# Autodesk Inventor assembly: Jar Jar
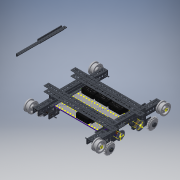
[picture p0: Inventor's stored thumbnail of the model, 180x180]
Saved by Autodesk Inventor 2016 (Build 200138000, 138)
## iProperties
Created: 2015-12-13
Part Number: Jar Jar
Document SubType Name: Assembly
Designer: tbloo
Author: tbloo
## Documents named in this file (19)
- C:\Users\TimB\Documents\GitHub\phi_robotics\3d-models\FTC_Tetrix_KOP_Block_Party\Tim Bloot Designs\JAr JaR Bot\Jar Jar.iam
- C:\Users\TimB\Documents\GitHub\phi_robotics\3d-models\FTC_Tetrix_KOP_Block_Party\Tim Bloot Designs\Base Plate.ipt
- C:\Users\TimB\Documents\GitHub\phi_robotics\3d-models\FTC_Tetrix_KOP_Block_Party\Tetrix_Kit_FTC\Autodesk Inventor Files\tetrix_c_channel-3.ipt
- C:\Users\TimB\Documents\GitHub\phi_robotics\3d-models\FTC_Tetrix_KOP_Block_Party\Tetrix_Kit_FTC\Autodesk Inventor Files\tetrix_c_channel-2.ipt
- C:\Users\TimB\Documents\GitHub\phi_robotics\3d-models\FTC_Tetrix_KOP_Block_Party\Tetrix_Kit_FTC\Autodesk Inventor Files\tetrix_motor_mount-old.ipt
- C:\Users\TimB\Documents\GitHub\phi_robotics\3d-models\FTC_Tetrix_KOP_Block_Party\Tetrix_Kit_FTC\Autodesk Inventor Files\tetrix_motor.iam
- C:\Users\TimB\Documents\GitHub\phi_robotics\3d-models\FTC_Tetrix_KOP_Block_Party\Tetrix_Kit_FTC\Autodesk Inventor Files\tetrix_bushing.ipt
- C:\Users\TimB\Documents\GitHub\phi_robotics\3d-models\FTC_Tetrix_KOP_Block_Party\Tim Bloot Designs\JAr JaR Bot\Tread Wheel Assembly.iam
- C:\Users\TimB\Documents\GitHub\phi_robotics\3d-models\FTC_Tetrix_KOP_Block_Party\Tetrix_Kit_FTC\Autodesk Inventor Files\tetrix_c_channel-5.ipt
- C:\Users\TimB\Documents\GitHub\phi_robotics\3d-models\FTC_Tetrix_KOP_Block_Party\Tetrix_Kit_FTC\Autodesk Inventor Files\tetrix_inside_corner_bracket.ipt
- C:\Users\TimB\Documents\GitHub\phi_robotics\3d-models\FTC_Tetrix_KOP_Block_Party\Tetrix_Kit_FTC\Autodesk Inventor Files\tetrix_motor_controller.ipt
- C:\Users\TimB\Documents\GitHub\phi_robotics\3d-models\FTC_Tetrix_KOP_Block_Party\Tetrix_Kit_FTC\Autodesk Inventor Files\tetrix_servo_controller.ipt
- C:\Users\TimB\Documents\GitHub\phi_robotics\3d-models\FTC_Tetrix_KOP_Block_Party\Tetrix_Kit_FTC\Autodesk Inventor Files\tetrix_c_channel-round.ipt
- C:\Users\TimB\Documents\GitHub\phi_robotics\3d-models\FTC_Tetrix_KOP_Block_Party\Tetrix_Kit_FTC\Autodesk Inventor Files\tetrix_c_channel-1.ipt
- C:\Users\TimB\Documents\GitHub\phi_robotics\3d-models\FTC_Tetrix_KOP_Block_Party\Tetrix_Kit_FTC\Autodesk Inventor Files\tetrix_angle-288 MM.ipt
- C:\Users\TimB\Documents\GitHub\phi_robotics\3d-models\FTC_Tetrix_KOP_Block_Party\Tim Bloot Designs\JAr JaR Bot\Tread Sproket Gear Assembly 2.iam
- C:\Users\TimB\Documents\GitHub\phi_robotics\3d-models\FTC_Tetrix_KOP_Block_Party\Tetrix_Kit_FTC\Autodesk Inventor Files\tetrix_739274_2013.ipt
- C:\Users\TimB\Documents\GitHub\phi_robotics\3d-models\FTC_Tetrix_KOP_Block_Party\Tim Bloot Designs\JAr JaR Bot\Motor Med Chain gear.iam
- C:\Users\TimB\Documents\GitHub\phi_robotics\3d-models\FTC_Tetrix_KOP_Block_Party\Tetrix_Kit_FTC\Autodesk Inventor Files\tetrix_angle-144 MM.ipt
## Components (61 placed, 18 different names)
1. Base Plate:1 — Rigid:60, Rigid:61, Rigid:63, Rigid:85, Rigid:108
2. tetrix_c_channel-3:4 — Rigid:55, Rigid:56, Rigid:76, Rigid:110
3. tetrix_c_channel-2:13 — Rigid:64, Rigid:86, Rigid:111
4. tetrix_c_channel-2:15 — Rigid:109
5. tetrix_c_channel-2:16
6. tetrix_motor_mount-old:6
7. tetrix_motor:5 [sub-assembly] — Rigid:91
8. Tread Wheel Assembly:5 [sub-assembly]
9. Tread Wheel Assembly:6 [sub-assembly]
10. tetrix_c_channel-5:1 — Rigid:55
11. tetrix_c_channel-5:2 — Rigid:59
12. tetrix_inside_corner_bracket:2 — Rigid:56, Rigid:59
13. tetrix_motor_controller:1 — Rigid:61, Rigid:62
14. tetrix_motor_controller:2 — Rigid:60
15. tetrix_motor_controller:3 — Rigid:62
16. tetrix_servo_controller:1 — Rigid:63
17. tetrix_c_channel-round:1 — Rigid:64, Rigid:65
18. tetrix_c_channel-1:1 — Rigid:65, Rotational:33, Rotational:34
19. tetrix_bushing:13 — Rotational:33, Rotational:42
20. tetrix_bushing:14 — Rotational:34
21. tetrix_c_channel-2:18 — Rigid:75
22. tetrix_motor_mount-old:8 — Rotational:41
23. tetrix_c_channel-round:3
24. tetrix_c_channel-1:3
25. tetrix_bushing:17
26. tetrix_bushing:18 — Rotational:43
27. tetrix_angle-288 MM:2 — Rigid:75, Rigid:76, Rigid:85, Rigid:86
28. tetrix_motor:6 [sub-assembly] — Rotational:41, Rigid:92
29. Tread Sproket Gear Assembly 2:1 [sub-assembly] — Rotational:42
30. Tread Sproket Gear Assembly 2:2 [sub-assembly] — Rotational:43
31. Motor Med Chain gear:1 [sub-assembly] — Rigid:92
32. Motor Med Chain gear:2 [sub-assembly] — Rigid:91
33. tetrix_c_channel-3:5
34. tetrix_c_channel-2:19
35. tetrix_c_channel-2:20
36. tetrix_c_channel-2:21
37. tetrix_motor_mount-old:9
38. tetrix_motor:7 [sub-assembly]
39. Tread Wheel Assembly:7 [sub-assembly]
40. Tread Wheel Assembly:8 [sub-assembly]
41. tetrix_c_channel-round:4
42. tetrix_c_channel-1:4
43. tetrix_bushing:19
44. tetrix_bushing:20
45. tetrix_c_channel-2:22
46. tetrix_motor_mount-old:10
47. tetrix_c_channel-round:5
48. tetrix_c_channel-1:5
49. tetrix_bushing:21
50. tetrix_bushing:22
51. tetrix_angle-288 MM:3 — Rigid:108
52. tetrix_motor:8 [sub-assembly]
53. Tread Sproket Gear Assembly 2:3 [sub-assembly]
54. Tread Sproket Gear Assembly 2:4 [sub-assembly]
55. tetrix_739274_2013:3
56. tetrix_739274_2013:4
57. Motor Med Chain gear:3 [sub-assembly]
58. Motor Med Chain gear:4 [sub-assembly]
59. tetrix_angle-288 MM:4
60. tetrix_angle-144 MM:1 — Rigid:109, Rigid:110, Rigid:111
61. tetrix_angle-144 MM:2
## Relationships (58: WeldJoint 38, RevoluteJoint 20)
- [WeldJoint]: tetrix_c_channel-2:13 ↔ tetrix_motor_mount-old:6
- [RevoluteJoint]: tetrix_motor_mount-old:6 ↔ tetrix_motor:5
- [RevoluteJoint]: tetrix_c_channel-2:15 ↔ Tread Wheel Assembly:5
- [RevoluteJoint]: tetrix_c_channel-2:16 ↔ Tread Wheel Assembly:6
- Rigid:55 [WeldJoint]: tetrix_c_channel-3:4 ↔ tetrix_c_channel-5:1
- Rigid:56 [WeldJoint]: tetrix_c_channel-3:4 ↔ tetrix_inside_corner_bracket:2
- Rigid:59 [WeldJoint]: tetrix_c_channel-5:2 ↔ tetrix_inside_corner_bracket:2
- Rigid:60 [WeldJoint]: Base Plate:1 ↔ tetrix_motor_controller:2
- Rigid:61 [WeldJoint]: Base Plate:1 ↔ tetrix_motor_controller:1
- Rigid:62 [WeldJoint]: tetrix_motor_controller:1 ↔ tetrix_motor_controller:3
- Rigid:63 [WeldJoint]: Base Plate:1 ↔ tetrix_servo_controller:1
- Rigid:64 [WeldJoint]: tetrix_c_channel-2:13 ↔ tetrix_c_channel-round:1
- Rigid:65 [WeldJoint]: tetrix_c_channel-round:1 ↔ tetrix_c_channel-1:1
- Rotational:33 [RevoluteJoint]: tetrix_c_channel-1:1 ↔ tetrix_bushing:13
- Rotational:34 [RevoluteJoint]: tetrix_c_channel-1:1 ↔ tetrix_bushing:14
- [WeldJoint]: tetrix_c_channel-2:18 ↔ tetrix_motor_mount-old:8
- [WeldJoint]: tetrix_c_channel-2:18 ↔ tetrix_c_channel-round:3
- [WeldJoint]: tetrix_c_channel-round:3 ↔ tetrix_c_channel-1:3
- [RevoluteJoint]: tetrix_c_channel-1:3 ↔ tetrix_bushing:17
- [RevoluteJoint]: tetrix_c_channel-1:3 ↔ tetrix_bushing:18
- Rigid:75 [WeldJoint]: tetrix_c_channel-2:18 ↔ tetrix_angle-288 MM:2
- Rigid:76 [WeldJoint]: tetrix_c_channel-3:4 ↔ tetrix_angle-288 MM:2
- Rotational:41 [RevoluteJoint]: tetrix_motor_mount-old:8 ↔ tetrix_motor:6
- Rotational:42 [RevoluteJoint]: tetrix_bushing:13 ↔ Tread Sproket Gear Assembly 2:1
- Rotational:43 [RevoluteJoint]: tetrix_bushing:18 ↔ Tread Sproket Gear Assembly 2:2
- Rigid:85 [WeldJoint]: Base Plate:1 ↔ tetrix_angle-288 MM:2
- Rigid:86 [WeldJoint]: tetrix_c_channel-2:13 ↔ tetrix_angle-288 MM:2
- Rigid:91 [WeldJoint]: tetrix_motor:5 ↔ Motor Med Chain gear:2
- Rigid:92 [WeldJoint]: tetrix_motor:6 ↔ Motor Med Chain gear:1
- [WeldJoint]: tetrix_c_channel-2:19 ↔ tetrix_motor_mount-old:9
- [RevoluteJoint]: tetrix_motor_mount-old:9 ↔ tetrix_motor:7
- [RevoluteJoint]: tetrix_c_channel-2:20 ↔ Tread Wheel Assembly:7
- [RevoluteJoint]: tetrix_c_channel-2:21 ↔ Tread Wheel Assembly:8
- [WeldJoint]: tetrix_c_channel-2:19 ↔ tetrix_c_channel-round:4
- [WeldJoint]: tetrix_c_channel-round:4 ↔ tetrix_c_channel-1:4
- [RevoluteJoint]: tetrix_c_channel-1:4 ↔ tetrix_bushing:19
- [RevoluteJoint]: tetrix_c_channel-1:4 ↔ tetrix_bushing:20
- [WeldJoint]: tetrix_c_channel-2:22 ↔ tetrix_motor_mount-old:10
- [WeldJoint]: tetrix_c_channel-2:22 ↔ tetrix_c_channel-round:5
- [WeldJoint]: tetrix_c_channel-round:5 ↔ tetrix_c_channel-1:5
- [RevoluteJoint]: tetrix_c_channel-1:5 ↔ tetrix_bushing:21
- [RevoluteJoint]: tetrix_c_channel-1:5 ↔ tetrix_bushing:22
- [WeldJoint]: tetrix_c_channel-2:22 ↔ tetrix_angle-288 MM:3
- [WeldJoint]: tetrix_c_channel-3:5 ↔ tetrix_angle-288 MM:3
- [RevoluteJoint]: tetrix_motor_mount-old:10 ↔ tetrix_motor:8
- [RevoluteJoint]: tetrix_bushing:19 ↔ Tread Sproket Gear Assembly 2:3
- [RevoluteJoint]: tetrix_bushing:22 ↔ Tread Sproket Gear Assembly 2:4
- [WeldJoint]: tetrix_c_channel-2:19 ↔ tetrix_angle-288 MM:3
- [WeldJoint]: tetrix_c_channel-2:19 ↔ tetrix_739274_2013:3
- [WeldJoint]: tetrix_c_channel-2:20 ↔ tetrix_739274_2013:3
- [WeldJoint]: tetrix_c_channel-2:22 ↔ tetrix_739274_2013:4
- [WeldJoint]: tetrix_c_channel-2:21 ↔ tetrix_739274_2013:4
- [WeldJoint]: tetrix_motor:7 ↔ Motor Med Chain gear:4
- [WeldJoint]: tetrix_motor:8 ↔ Motor Med Chain gear:3
- Rigid:108 [WeldJoint]: Base Plate:1 ↔ tetrix_angle-288 MM:3
- Rigid:109 [WeldJoint]: tetrix_c_channel-2:15 ↔ tetrix_angle-144 MM:1
- Rigid:110 [WeldJoint]: tetrix_c_channel-3:4 ↔ tetrix_angle-144 MM:1
- Rigid:111 [WeldJoint]: tetrix_c_channel-2:13 ↔ tetrix_angle-144 MM:1
## Named parameters: d112_d58_d39 = 0 mm, d113_d59_d40 = -5.431137 deg, d114_d60_d41 = 0 mm, d115_d61_d42 = 0.840635 deg, d116_d65_d11 = 0 mm, d122_d71_d21 = 0 mm, d123_d72_d22 = -45.624239 deg, d153_d150_d116_d65_d11 = 0 mm, d154_d143_d137 = 0 mm, d155_d144_d138 = 0 mm, d156_d145_d139 = 0 mm, d157_d146_d140 = 0 deg, d158_d147_d141 = 0 mm, d159_d148_d142 = 0 deg, d210_d112_d58_d39 = 0 mm, d211_d113_d59_d40 = -5.431137 deg, d212_d170 = 0 mm, d213_d171 = 0 deg, d214_d203 = 0 mm, d215_d204 = 0 mm, d216_d205 = 0 mm, d217_d206 = 0 mm, d218_d207 = 0 mm, d219_d208 = 0 mm, d220_d209 = 0 mm, d221_d137 = 0 mm, d222_d138 = 0 mm, d223_d139 = 0 mm, d224_d140 = 0.202797 deg, d225_d141 = 0 mm, d226_d142 = 0 deg, d227_d153_d150_d116_d65_d11 = 0 mm, d228_d154_d143_d137 = 0 mm, d229_d155_d144_d138 = 0 mm, d230_d156_d145_d139 = 0 mm, d231_d157_d146_d140 = 0 deg, d232_d158_d147_d141 = 0 mm, d233_d159_d148_d142 = 0 deg, d234_d164 = 0 mm, d235_d165 = 0 mm, d236_d166 = 0 mm, d237_d167 = -134.685077 deg, d238_d168 = 0 mm, d239_d169 = -0.202797 deg, d240_d114_d60_d41 = 0 mm, d241_d115_d61_d42 = 0.840635 deg, d242_d116_d65_d11 = 0 mm, d243_d122_d71_d21 = 0 mm, d244_d123_d72_d22 = -50.322066 deg
